# Autodesk Inventor assembly: Desain3D
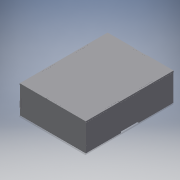
[picture p0: Inventor's stored thumbnail of the model, 180x180]
Saved by Autodesk Inventor 2017 (Build 210142000, 142)
## iProperties
Created: 2017-01-17
Part Number: Desain3D
Document SubType Name: Assembly
Designer: Ghesa Bhakti
Author: Ghesa Bhakti
## Documents named in this file (8)
- D:\RPL\Intel Atom\Desain 3D\Desain3D.iam
- D:\RPL\Intel Atom\Desain 3D\belakang.ipt
- D:\RPL\Intel Atom\Desain 3D\bawah.ipt
- D:\RPL\Intel Atom\Desain 3D\atas.ipt
- D:\RPL\Intel Atom\Desain 3D\sampingkanan.ipt
- D:\RPL\Intel Atom\Desain 3D\sampingkiri.ipt
- D:\RPL\Intel Atom\Desain 3D\depan.ipt
- D:\RPL\Intel Atom\Desain 3D\kunci.ipt
## Components (7 placed, 7 different names)
1. belakang:1 — Angle:1, Mate:1, Angle:2, Mate:2, Angle:3, Mate:3, Angle:5, Mate:4
2. bawah:1 — Angle:1, Mate:1
3. atas:1 — Angle:2, Mate:2, Angle:4, Mate:6
4. sampingkanan:1 — Angle:3, Angle:4, Mate:3, Mate:5
5. sampingkiri:1 — Angle:5, Mate:4, Mate:7, Mate:8
6. depan:1 — Mate:5, Mate:6
7. kunci:1 — Mate:7, Mate:8
## Relationships (13: Mate 8, Angle 5)
- Angle:1 (90 deg): belakang:1 ↔ bawah:1
- Mate:1: belakang:1 ↔ bawah:1
- Angle:2 (90 deg): belakang:1 ↔ atas:1
- Mate:2: belakang:1 ↔ atas:1
- Angle:3 (90 deg): belakang:1 ↔ sampingkanan:1
- Angle:4 (180 deg): atas:1 ↔ sampingkanan:1
- Mate:3: belakang:1 ↔ sampingkanan:1
- Angle:5 (90 deg): belakang:1 ↔ sampingkiri:1
- Mate:4: belakang:1 ↔ sampingkiri:1
- Mate:5: sampingkanan:1 ↔ depan:1
- Mate:6: atas:1 ↔ depan:1
- Mate:7: sampingkiri:1 ↔ kunci:1
- Mate:8: sampingkiri:1 ↔ kunci:1
